# Autodesk Inventor assembly: 276-2185
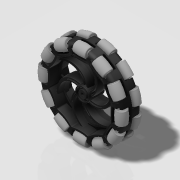
[picture p0: Inventor's stored thumbnail of the model, 180x180]
Saved by Autodesk Inventor 2021 (Build 250183000, 183)
## iProperties
Part Number: 276-2185
Document SubType Name: Assembly
Designer: Jordan Kiesel
Mass: 105.233 g
Surface Area: 931.315 cm^2
Volume: 89.3073 cm^3
Catalog Web Link: vexrobotics.com/276-2185.html
Description: Roll forward like normal wheels, but slide sideways with almost no friction.
Vendor: VEX Robotics, Inc.
Density: 1.17833 g/cm^3
Created: 2019-06-10
Category: Motion
Company: Super Sonic Sparks, Team 24
Translation Standard: STEP AP203
FileName: 4'' Omni-Directional Wheel.iam
PreProcessor: SolidWorks 2006052
PostProcessor: Build: 239, Release: 2011 RTM - Date: Wed 02/17/2010
Sent Units: inch
Uncertainty: 1e-05
Author: Jordan Kiesel
Title: 4" Omni-Directional Wheel
Comments: Omni-Directional wheels roll forward like normal wheels, but slide sideways with almost no friction (no skidding during turns). Use these wheels to make your robot turn smoothly or build a holonomic drivetrain. These wheels are the same size as the VEX 4" dia. Wheels. ▷ 4" Omni Wheels roll sideways with very little friction. ▷ Minimize skidding during turns. ▷ Build a holonomic drive.
## Documents named in this file (4)
- E:\VEX Library\Motion\Wheels _ Rollers\4 Omni.iam
- E:\VEX Library\Motion\Wheels _ Rollers\Reference Parts\4_ Omni-Directional Wheel\Roller.iam
- E:\VEX Library\Motion\Wheels _ Rollers\Reference Parts\4_ Omni-Directional Wheel\Hub Insert.ipt
- E:\VEX Library\Motion\Wheels _ Rollers\Reference Parts\4_ Omni-Directional Wheel\Hub.ipt
## Components (26 placed, 3 different names)
1. Hub:1 — Mate:1, Mate:2, Mate:3, Mate:4, Mate:5, Mate:6, Mate:7, Mate:8, Mate:9, Mate:10, Mate:11, Mate:12, Mate:13, Mate:14, Mate:15, Mate:16, Mate:17, Mate:18, Mate:19, Mate:20, Mate:21, Mate:22, Mate:23, Mate:24, Mate:25, Mate:26, Mate:27, Mate:28, Mate:29, Mate:30, Mate:31, Mate:32, Mate:33, Mate:34, Mate:35, Mate:36, Mate:37, Mate:38, Mate:39, Mate:40, Mate:41, Mate:42, Mate:43, Mate:44, Mate:45, Mate:46, Mate:47, Mate:48
2. Hub Insert:1
3. Roller:1 [sub-assembly] — Mate:1, Mate:2
4. Roller:2 [sub-assembly] — Mate:3, Mate:4
5. Roller:3 [sub-assembly] — Mate:5, Mate:6
6. Roller:4 [sub-assembly] — Mate:7, Mate:8
7. Roller:5 [sub-assembly] — Mate:9, Mate:10
8. Roller:6 [sub-assembly] — Mate:11, Mate:12
9. Roller:7 [sub-assembly] — Mate:13, Mate:14
10. Roller:8 [sub-assembly] — Mate:15, Mate:16
11. Roller:9 [sub-assembly] — Mate:17, Mate:18
12. Roller:10 [sub-assembly] — Mate:19, Mate:20
13. Roller:11 [sub-assembly] — Mate:21, Mate:22
14. Roller:12 [sub-assembly] — Mate:23, Mate:24
15. Roller:13 [sub-assembly] — Mate:25, Mate:26
16. Roller:14 [sub-assembly] — Mate:27, Mate:28
17. Roller:15 [sub-assembly] — Mate:29, Mate:30
18. Roller:16 [sub-assembly] — Mate:31, Mate:32
19. Roller:17 [sub-assembly] — Mate:33, Mate:34
20. Roller:18 [sub-assembly] — Mate:35, Mate:36
21. Roller:19 [sub-assembly] — Mate:37, Mate:38
22. Roller:20 [sub-assembly] — Mate:39, Mate:40
23. Roller:21 [sub-assembly] — Mate:41, Mate:42
24. Roller:22 [sub-assembly] — Mate:43, Mate:44
25. Roller:23 [sub-assembly] — Mate:45, Mate:46
26. Roller:24 [sub-assembly] — Mate:47, Mate:48
## Relationships (48: Mate 48)
- Mate:1: Hub:1 ↔ Roller:1
- Mate:2 (0.308 mm): Hub:1 ↔ Roller:1
- Mate:3: Hub:1 ↔ Roller:2
- Mate:4 (0.308 mm): Hub:1 ↔ Roller:2
- Mate:5: Hub:1 ↔ Roller:3
- Mate:6 (0.308 mm): Hub:1 ↔ Roller:3
- Mate:7: Hub:1 ↔ Roller:4
- Mate:8 (0.308 mm): Hub:1 ↔ Roller:4
- Mate:9: Hub:1 ↔ Roller:5
- Mate:10 (0.308 mm): Hub:1 ↔ Roller:5
- Mate:11: Hub:1 ↔ Roller:6
- Mate:12 (0.308 mm): Hub:1 ↔ Roller:6
- Mate:13: Hub:1 ↔ Roller:7
- Mate:14 (0.308 mm): Hub:1 ↔ Roller:7
- Mate:15: Hub:1 ↔ Roller:8
- Mate:16 (0.308 mm): Hub:1 ↔ Roller:8
- Mate:17: Hub:1 ↔ Roller:9
- Mate:18 (0.308 mm): Hub:1 ↔ Roller:9
- Mate:19: Hub:1 ↔ Roller:10
- Mate:20 (0.308 mm): Hub:1 ↔ Roller:10
- Mate:21: Hub:1 ↔ Roller:11
- Mate:22 (0.308 mm): Hub:1 ↔ Roller:11
- Mate:23: Hub:1 ↔ Roller:12
- Mate:24 (0.308 mm): Hub:1 ↔ Roller:12
- Mate:25: Hub:1 ↔ Roller:13
- Mate:26 (0.308 mm): Hub:1 ↔ Roller:13
- Mate:27: Hub:1 ↔ Roller:14
- Mate:28 (0.308 mm): Hub:1 ↔ Roller:14
- Mate:29: Hub:1 ↔ Roller:15
- Mate:30 (0.308 mm): Hub:1 ↔ Roller:15
- Mate:31: Hub:1 ↔ Roller:16
- Mate:32 (0.308 mm): Hub:1 ↔ Roller:16
- Mate:33: Hub:1 ↔ Roller:17
- Mate:34 (0.308 mm): Hub:1 ↔ Roller:17
- Mate:35: Hub:1 ↔ Roller:18
- Mate:36 (0.308 mm): Hub:1 ↔ Roller:18
- Mate:37: Hub:1 ↔ Roller:19
- Mate:38 (0.308 mm): Hub:1 ↔ Roller:19
- Mate:39: Hub:1 ↔ Roller:20
- Mate:40 (0.308 mm): Hub:1 ↔ Roller:20
- Mate:41: Hub:1 ↔ Roller:21
- Mate:42 (0.308 mm): Hub:1 ↔ Roller:21
- Mate:43: Hub:1 ↔ Roller:22
- Mate:44 (0.308 mm): Hub:1 ↔ Roller:22
- Mate:45: Hub:1 ↔ Roller:23
- Mate:46 (0.308 mm): Hub:1 ↔ Roller:23
- Mate:47: Hub:1 ↔ Roller:24
- Mate:48 (0.308 mm): Hub:1 ↔ Roller:24
